# Autodesk Inventor assembly: Ensamblaje_Mesa
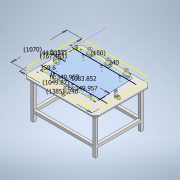
[picture p0: Inventor's stored thumbnail of the model, 180x180]
Saved by Autodesk Inventor 2021 (Build 250183000, 183)
## iProperties
Created: 2021-06-07
Part Number: Ensamblaje_Mesa
Document SubType Name: Assembly
Designer: Mecatronica
Author: Mecatronica
## Documents named in this file (8)
- G:\Unidades compartidas\Robótica\Proyecto\Ensamblaje_Mesa_vidrio.iam
- G:\Unidades compartidas\Robótica\Proyecto\Mesa_Centrado.ipt
- G:\Unidades compartidas\Robótica\Proyecto\Ventanas.ipt
- G:\Unidades compartidas\Robótica\Proyecto\Rodillo1.ipt
- G:\Unidades compartidas\Robótica\Proyecto\Rodillo2.ipt
- G:\Unidades compartidas\Robótica\Proyecto\Rodillo3.ipt
- G:\Unidades compartidas\Robótica\Proyecto\Rodillo_Sostener.ipt
- G:\Unidades compartidas\Robótica\Proyecto\Riel.ipt
## Components (20 placed, 7 different names)
1. Mesa_Centrado:1 — Coincidencia:3, Coincidencia:4, Coincidencia:5, Coincidencia:6, Coincidencia:7, Coincidencia:8, Tangente:3, Tangente:4, Tangente:6, Tangente:7, Tangente:8, Tangente:9, Tangente:10, Tangente:11, Tangente:12, Tangente:13, Tangente:14, Tangente:15, Coincidencia:9, Coincidencia:10, Coincidencia:11, Coincidencia:12, Tangente:16, Nivelación:2, Nivelación:3, Nivelación:4, Tangente:17, Tangente:18, Nivelación:5, Tangente:19, Coincidencia:13, Tangente:20, Nivelación:6, Coincidencia:14, Nivelación:7, Tangente:21, Nivelación:8
2. Ventanas:1 — Nivelación:8
3. Rodillo1:1 — Insertar:3
4. Rodillo1:2 — Insertar:2
5. Rodillo1:3 — Insertar:1
6. Rodillo2:1 — Insertar:6
7. Rodillo2:2 — Insertar:5
8. Rodillo3:1 — Insertar:4
9. Rodillo_Sostener:1 — Coincidencia:7, Tangente:10, Tangente:11
10. Rodillo_Sostener:2 — Coincidencia:8, Tangente:8, Tangente:9
11. Rodillo_Sostener:3 — Coincidencia:6, Tangente:6, Tangente:7
12. Rodillo_Sostener:4 — Coincidencia:3, Tangente:3, Tangente:4
13. Rodillo_Sostener:5 — Coincidencia:5, Tangente:12, Tangente:14
14. Rodillo_Sostener:6 — Coincidencia:4, Tangente:13, Tangente:15
15. Riel:1 — Coincidencia:9, Nivelación:5, Tangente:19, Insertar:6
16. Riel:2 — Coincidencia:10, Tangente:16, Nivelación:2, Insertar:1
17. Riel:3 — Coincidencia:11, Nivelación:3, Tangente:17, Insertar:2
18. Riel:4 — Coincidencia:12, Nivelación:4, Tangente:18, Insertar:3
19. Riel:5 — Coincidencia:13, Tangente:20, Nivelación:6, Insertar:5
20. Riel:6 — Coincidencia:14, Nivelación:7, Tangente:21, Insertar:4
## Relationships (43: Tangent 18, Mate 12, Flush 7, Insert 6)
- Coincidencia:3 [Mate]: Mesa_Centrado:1 ↔ Rodillo_Sostener:4
- Coincidencia:4 [Mate]: Mesa_Centrado:1 ↔ Rodillo_Sostener:6
- Coincidencia:5 [Mate]: Mesa_Centrado:1 ↔ Rodillo_Sostener:5
- Coincidencia:6 [Mate]: Mesa_Centrado:1 ↔ Rodillo_Sostener:3
- Coincidencia:7 [Mate]: Mesa_Centrado:1 ↔ Rodillo_Sostener:1
- Coincidencia:8 [Mate]: Mesa_Centrado:1 ↔ Rodillo_Sostener:2
- Tangente:3 (344.5996 mm): Mesa_Centrado:1 ↔ Rodillo_Sostener:4
- Tangente:4 (225 mm): Mesa_Centrado:1 ↔ Rodillo_Sostener:4
- Tangente:6 (-255 mm): Mesa_Centrado:1 ↔ Rodillo_Sostener:3
- Tangente:7 (694.5561 mm): Mesa_Centrado:1 ↔ Rodillo_Sostener:3
- Tangente:8 (225 mm): Mesa_Centrado:1 ↔ Rodillo_Sostener:2
- Tangente:9 (1044.5127 mm): Mesa_Centrado:1 ↔ Rodillo_Sostener:2
- Tangente:10 (344.5996 mm): Mesa_Centrado:1 ↔ Rodillo_Sostener:1
- Tangente:11 (225 mm): Mesa_Centrado:1 ↔ Rodillo_Sostener:1
- Tangente:12 (225 mm): Mesa_Centrado:1 ↔ Rodillo_Sostener:5
- Tangente:13 (225 mm): Mesa_Centrado:1 ↔ Rodillo_Sostener:6
- Tangente:14 (694.5561 mm): Mesa_Centrado:1 ↔ Rodillo_Sostener:5
- Tangente:15 (1044.5127 mm): Mesa_Centrado:1 ↔ Rodillo_Sostener:6
- Coincidencia:9 [Mate]: Mesa_Centrado:1 ↔ Riel:1
- Coincidencia:10 [Mate]: Mesa_Centrado:1 ↔ Riel:2
- Coincidencia:11 [Mate]: Mesa_Centrado:1 ↔ Riel:3
- Coincidencia:12 [Mate]: Mesa_Centrado:1 ↔ Riel:4
- Tangente:16 (-133.3333 mm): Mesa_Centrado:1 ↔ Riel:2
- Nivelación:2 [Flush] (1037.8461 mm): Mesa_Centrado:1 ↔ Riel:2
- Nivelación:3 [Flush] (687.8895 mm): Mesa_Centrado:1 ↔ Riel:3
- Nivelación:4 [Flush] (337.9329 mm): Mesa_Centrado:1 ↔ Riel:4
- Tangente:17 (-133.3333 mm): Mesa_Centrado:1 ↔ Riel:3
- Tangente:18 (-133.3333 mm): Mesa_Centrado:1 ↔ Riel:4
- Nivelación:5 [Flush] (-513.3333 mm): Mesa_Centrado:1 ↔ Riel:1
- Tangente:19 (-150.786 mm): Mesa_Centrado:1 ↔ Riel:1
- Coincidencia:13 [Mate]: Mesa_Centrado:1 ↔ Riel:5
- Tangente:20 (-133.3333 mm): Mesa_Centrado:1 ↔ Riel:5
- Nivelación:6 [Flush] (-687.8895 mm): Mesa_Centrado:1 ↔ Riel:5
- Coincidencia:14 [Mate]: Mesa_Centrado:1 ↔ Riel:6
- Nivelación:7 [Flush] (513.3333 mm): Mesa_Centrado:1 ↔ Riel:6
- Tangente:21 (-159.1193 mm): Mesa_Centrado:1 ↔ Riel:6
- Nivelación:8 [Flush] (150 mm): Mesa_Centrado:1 ↔ Ventanas:1
- Insertar:1: Rodillo1:3 ↔ Riel:2
- Insertar:2: Rodillo1:2 ↔ Riel:3
- Insertar:3: Rodillo1:1 ↔ Riel:4
- Insertar:4: Rodillo3:1 ↔ Riel:6
- Insertar:5: Rodillo2:2 ↔ Riel:5
- Insertar:6: Rodillo2:1 ↔ Riel:1
